# Autodesk Inventor assembly: Rstove
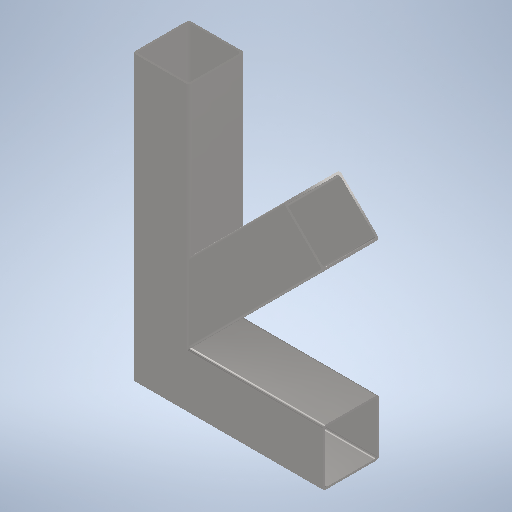
[picture p0: Inventor's stored thumbnail of the model, 512x512]
Saved by Autodesk Inventor 2025.2 (Build 292293000, 293)
## iProperties
Created: 2025-04-08
Part Number: Rstove
Document SubType Name: Assembly
Designer: bless
Author: bless
## Documents named in this file (3)
- C:\Users\bless\OneDrive - Conestoga College\Documents\Inventor\8071W25\Rstove\Rstove.iam
- C:\Users\bless\OneDrive - Conestoga College\Documents\Inventor\8071W25\Rstove\6527K433_Low-Carbon Steel Rectangular Tube\6527K433_Low-Carbon Steel Rectangular Tube\6527K433_Low-Carbon Steel Rectangular Tube.ipt
- C:\Users\bless\OneDrive - Conestoga College\Documents\Inventor\8071W25\Rstove\6527K433_Low-Carbon Steel Rectangular Tube\6527K433_Low-Carbon Steel Rectangular Tube\base.ipt
## Components (3 placed, 2 different names)
1. 6527K433_Low-Carbon Steel Rectangular Tube:1 — Flush:1, Mate:1, Flush:2
2. base:2 — Mate:1, Flush:2, Mate:2
3. base:1 — Mate:2
## Component patterns: (2 elements, first: base:1)
## Relationships (4: Flush 2, Mate 2)
- Flush:1: 6527K433_Low-Carbon Steel Rectangular Tube:1
- Mate:1: 6527K433_Low-Carbon Steel Rectangular Tube:1 ↔ base:2
- Flush:2: 6527K433_Low-Carbon Steel Rectangular Tube:1 ↔ base:2
- Mate:2: base:2 ↔ base:1
